# Autodesk Inventor assembly: +XPanel
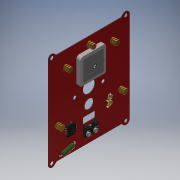
[picture p0: Inventor's stored thumbnail of the model, 180x180]
Saved by Autodesk Inventor 2018 (Build 220112000, 112)
## iProperties
Created: 2018-10-25
Part Number: +XPanel
Document SubType Name: Assembly
Designer: Bradley
Author: Bradley
## Documents named in this file (13)
- C:\Users\Bradley\Documents\GitHub\CougSat1-Hardware\CougSat1-RadioBoard\CADModel\Native\+XPanel.iam
- C:\Users\Bradley\Documents\GitHub\CougSat1-Hardware\CougSat1-RadioBoard\CADModel\Native\+XPanel_PCB.ipt
- C:\Users\Bradley\Documents\GitHub\Resources\ComponentModels\Electronics\Antenna_GPSPatch.ipt
- C:\Users\Bradley\Documents\GitHub\Resources\ComponentModels\Connectors\PinRecepticle-0.38-0.56mm.ipt
- C:\Users\Bradley\Documents\GitHub\Resources\ComponentModels\Connectors\U.FL_Male.ipt
- C:\Users\Bradley\Documents\GitHub\Resources\ComponentModels\Electronics\Resistor_TH-15mm.ipt
- C:\Users\Bradley\Documents\GitHub\CougSat1-Hardware\CougSat1-RadioBoard\CADModel\Native\+XPanel_AntennaPost.ipt
- C:\Users\Bradley\Documents\GitHub\Resources\ComponentModels\Fasteners\Bolt_M2x0.4_4mm_SH.ipt
- C:\Users\Bradley\Documents\GitHub\Resources\ComponentModels\Fasteners\Nut_SMD_M2x0.4_1mm.ipt
- C:\Users\Bradley\Documents\GitHub\CougSat1-Hardware\CougSat1-RadioBoard\CADModel\Native\+XPanel_AntennaMount.ipt
- C:\Users\Bradley\Documents\GitHub\Resources\ComponentModels\Connectors\PicoLock-J-4.ipt
- C:\Users\Bradley\Documents\GitHub\Resources\ComponentModels\Connectors\PicoLock-P-4.ipt
- C:\Users\Bradley\Documents\GitHub\Resources\ComponentModels\Connectors\U.FL_Female.ipt
## Components (21 placed, 12 different names)
1. +XPanel_PCB:1 — Insert:1, Insert:2, Insert:3, Mate:1, Mate:2, Insert:4, Insert:5, Insert:6, Insert:7, Insert:8, Insert:9, Insert:10, Insert:11, Insert:12, Mate:5
2. Antenna_GPSPatch:1 — Insert:1, Flush:1
3. PinRecepticle-0.38-0.56mm:1 — Insert:3
4. PinRecepticle-0.38-0.56mm:2 — Insert:2
5. U.FL_Male:1 — Mate:1, Mate:7, Flush:4, Insert:16
6. U.FL_Male:2 — Mate:2, Flush:5, Mate:8, Insert:15
7. Resistor_TH-15mm:1
8. +XPanel_AntennaPost:1 — Insert:4
9. +XPanel_AntennaPost:2 — Insert:8
10. +XPanel_AntennaPost:3 — Insert:7
11. +XPanel_AntennaPost:4 — Insert:6
12. +XPanel_AntennaPost:5 — Insert:5
13. Bolt_M2x0.4_4mm_SH:1 — Insert:13
14. Nut_SMD_M2x0.4_1mm:1 — Insert:9
15. Nut_SMD_M2x0.4_1mm:2 — Insert:10
16. +XPanel_AntennaMount:1 — Insert:11, Insert:12, Insert:13, Insert:14
17. Bolt_M2x0.4_4mm_SH:2 — Insert:14
18. PicoLock-J-4:1 — Mate:5, Flush:3, Mate:6
19. PicoLock-P-4:1
20. U.FL_Female:1 — Insert:16, Angle:1
21. U.FL_Female:2 — Insert:15, Angle:2
## Relationships (31: Insert 16, Mate 8, Flush 5, Angle 2)
- Insert:1: +XPanel_PCB:1 ↔ Antenna_GPSPatch:1
- Flush:1: Antenna_GPSPatch:1
- Insert:2: +XPanel_PCB:1 ↔ PinRecepticle-0.38-0.56mm:2
- Insert:3: +XPanel_PCB:1 ↔ PinRecepticle-0.38-0.56mm:1
- Mate:1: +XPanel_PCB:1 ↔ U.FL_Male:1
- Mate:2: +XPanel_PCB:1 ↔ U.FL_Male:2
- Insert:4: +XPanel_PCB:1 ↔ +XPanel_AntennaPost:1
- Insert:5: +XPanel_PCB:1 ↔ +XPanel_AntennaPost:5
- Insert:6: +XPanel_PCB:1 ↔ +XPanel_AntennaPost:4
- Insert:7: +XPanel_PCB:1 ↔ +XPanel_AntennaPost:3
- Insert:8: +XPanel_PCB:1 ↔ +XPanel_AntennaPost:2
- Insert:9: +XPanel_PCB:1 ↔ Nut_SMD_M2x0.4_1mm:1
- Insert:10: +XPanel_PCB:1 ↔ Nut_SMD_M2x0.4_1mm:2
- Insert:11: +XPanel_PCB:1 ↔ +XPanel_AntennaMount:1
- Insert:12: +XPanel_PCB:1 ↔ +XPanel_AntennaMount:1
- Insert:13: Bolt_M2x0.4_4mm_SH:1 ↔ +XPanel_AntennaMount:1
- Insert:14: +XPanel_AntennaMount:1 ↔ Bolt_M2x0.4_4mm_SH:2
- [Flush]: PicoLock-J-4:1 ↔ PicoLock-P-4:1
- [Mate]: PicoLock-J-4:1 ↔ PicoLock-P-4:1
- [Mate] (0.025 mm): PicoLock-J-4:1 ↔ PicoLock-P-4:1
- Mate:5: +XPanel_PCB:1 ↔ PicoLock-J-4:1
- Flush:3 (23 mm): PicoLock-J-4:1
- Mate:6 (-24 mm): PicoLock-J-4:1
- Mate:7 (20 mm): U.FL_Male:1
- Flush:4 (20 mm): U.FL_Male:1
- Flush:5 (15 mm): U.FL_Male:2
- Mate:8 (20 mm): U.FL_Male:2
- Insert:15 (0.1 mm): U.FL_Male:2 ↔ U.FL_Female:2
- Insert:16 (0.1 mm): U.FL_Male:1 ↔ U.FL_Female:1
- Angle:1 (30 deg): U.FL_Female:1
- Angle:2 (30 deg): U.FL_Female:2
## Named parameters: d105_d9 = 0 mm, d106_d10 = 0 mm, d107_d11 = 0.025 mm
